# Autodesk Inventor assembly: EnglishAssembly
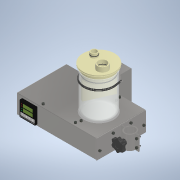
[picture p0: Inventor's stored thumbnail of the model, 180x180]
Saved by Autodesk Inventor 2020 (Build 240168000, 168)
## iProperties
Created: 2020-07-27
Part Number: EnglishAssembly
Document SubType Name: Assembly
Designer: Samuel
Author: Samuel
## Documents named in this file (31)
- C:\Users\Samuel\Desktop\EnglishAssembly.iam
- C:\Users\Samuel\Desktop\CNAF\CNAFgit\OpenHFNC\CAD\Prototype 3 (eng)\Box base_v7.ipt
- C:\Users\Samuel\Desktop\CNAF\CNAFgit\OpenHFNC\CAD\Prototype 3 (eng)\M4 Rivet nut.ipt
- C:\Users\Samuel\Desktop\CNAF\CNAFgit\OpenHFNC\CAD\Prototype 3 (eng)\RexC100 Temp control.ipt
- C:\Users\Samuel\Desktop\CNAF\CNAFgit\OpenHFNC\CAD\Prototype 3 (eng)\Switch OnOff 240V20A.ipt
- C:\Users\Samuel\Desktop\CNAF\CNAFgit\OpenHFNC\CAD\Prototype 3 (eng)\Solid State Rele SSR40DA.ipt
- C:\Users\Samuel\Desktop\CNAF\CNAFgit\OpenHFNC\CAD\Prototype 3 (eng)\Box top_v7.ipt
- C:\Users\Samuel\Desktop\CNAF\CNAFgit\OpenHFNC\CAD\Prototype 3 (eng)\Heater disk.ipt
- C:\Users\Samuel\Desktop\CNAF\CNAFgit\OpenHFNC\CAD\Prototype 3 (eng)\Oring 2-343.ipt
- C:\Users\Samuel\Desktop\CNAF\CNAFgit\OpenHFNC\CAD\Prototype 3 (eng)\Heater630W.ipt
- C:\Users\Samuel\Desktop\CNAF\CNAFgit\OpenHFNC\CAD\Prototype 3 (eng)\DIN912 M4x0.7x40-8.8 socket head screw.ipt
- C:\Users\Samuel\Desktop\CNAF\CNAFgit\OpenHFNC\CAD\Prototype 3 (eng)\DIN934-M4 nut.ipt
- C:\Users\Samuel\Desktop\CNAF\CNAFgit\OpenHFNC\CAD\Prototype 3 (eng)\DIN913-M5x5 socket screw flat end.ipt
- C:\Users\Samuel\Desktop\CNAF\CNAFgit\OpenHFNC\CAD\Prototype 3 (eng)\Thermocouple.ipt
- C:\Users\Samuel\Desktop\CNAF\CNAFgit\OpenHFNC\CAD\Prototype 3 (eng)\Heater Fixing Bar.ipt
- C:\Users\Samuel\Desktop\CNAF\CNAFgit\OpenHFNC\CAD\Prototype 3 (eng)\IEC C14 Male panel conector.ipt
- C:\Users\Samuel\Desktop\CNAF\CNAFgit\OpenHFNC\CAD\Prototype 3 (eng)\Precipitated Glass 600ml-De90-Di84-H120.ipt
- C:\Users\Samuel\Desktop\CNAF\CNAFgit\OpenHFNC\CAD\Prototype 3 (eng)\DIN912 M4x0.7x10-8.8 socket head screw.ipt
- C:\Users\Samuel\Desktop\CNAF\CNAFgit\OpenHFNC\CAD\Prototype 3 (eng)\DIN7991 M3x0.5x10-8.8 countersunk head cap screws.ipt
- C:\Users\Samuel\Desktop\CNAF\CNAFgit\OpenHFNC\CAD\Prototype 3 (eng)\Glass fixer plate.ipt
- C:\Users\Samuel\Desktop\CNAF\CNAFgit\OpenHFNC\CAD\Prototype 3 (eng)\Oring 2-159 Glass plate fixer.ipt
- C:\Users\Samuel\Desktop\CNAF\CNAFgit\OpenHFNC\CAD\Prototype 3 (eng)\Body glass top.ipt
- C:\Users\Samuel\Desktop\CNAF\CNAFgit\OpenHFNC\CAD\Prototype 3 (eng)\Oring 2-151 Deform.ipt
- C:\Users\Samuel\Desktop\CNAF\CNAFgit\OpenHFNC\CAD\Prototype 3 (eng)\DIN912 M4x0.7x16-8.8 socket head screw.ipt
- C:\Users\Samuel\Desktop\CNAF\CNAFgit\OpenHFNC\CAD\Prototype 3 (eng)\Corrugated-top connector.ipt
- C:\Users\Samuel\Desktop\CNAF\CNAFgit\OpenHFNC\CAD\Prototype 3 (eng)\Heated tube-top connector.ipt
- C:\Users\Samuel\Desktop\CNAF\CNAFgit\OpenHFNC\CAD\Prototype 3 (eng)\Oring 2-018 Deform.ipt
- C:\Users\Samuel\Desktop\CNAF\CNAFgit\OpenHFNC\CAD\Prototype 3 (eng)\Oring 2-022.ipt
- C:\Users\Samuel\Desktop\CNAF\CNAFgit\OpenHFNC\CAD\Prototype 3 (eng)\Paddle.ipt
- C:\Users\Samuel\Desktop\box-iv stand connector.iam
- C:\Users\Samuel\Desktop\CNAF\CNAFgit\OpenHFNC\CAD\Prototype 3 (eng)\Star Knob 1-4UNC.ipt
## Components (67 placed, 30 different names)
1. Box base_v7:1 — Cylindrical:1, Cylindrical:2, Cylindrical:3, Cylindrical:4, Cylindrical:5, Cylindrical:6, Cylindrical:7, Cylindrical:8, Rotational:1, Cylindrical:9, Rotational:2, Cylindrical:10, Cylindrical:11, Cylindrical:12, Rigid:1, Rigid:2, Rigid:3, Cylindrical:13, Rotational:7, Rotational:14
2. M4 Rivet nut:1 — Cylindrical:3
3. M4 Rivet nut:2 — Cylindrical:1
4. M4 Rivet nut:3 — Cylindrical:4
5. M4 Rivet nut:4 — Cylindrical:5
6. M4 Rivet nut:5 — Rotational:1
7. M4 Rivet nut:6 — Cylindrical:2
8. M4 Rivet nut:7 — Cylindrical:6
9. M4 Rivet nut:8 — Cylindrical:9
10. M4 Rivet nut:9 — Cylindrical:8
11. M4 Rivet nut:10 — Rotational:2
12. M4 Rivet nut:11 — Cylindrical:7
13. M4 Rivet nut:12 — Cylindrical:11
14. M4 Rivet nut:13 — Cylindrical:10
15. M4 Rivet nut:14 — Cylindrical:12
16. RexC100 Temp control:1 — Rigid:1
17. Switch OnOff 240V20A:1 — Rigid:2
18. SSR-XXDA:1 — Rigid:3
19. Box top_v7:1 — Cylindrical:13, Rotational:3, Cylindrical:15, Cylindrical:16, Cylindrical:20, Cylindrical:21, Rotational:9, Cylindrical:22, Cylindrical:23, Rotational:10, Rotational:11, Cylindrical:24, Rotational:17, Rotational:18, Cylindrical:30, Cylindrical:31
20. Heater disk:1 — Rotational:3, Rigid:4, Cylindrical:14, Rotational:4, Rotational:5, Cylindrical:17, Cylindrical:19, Rotational:8
21. Oring 2-343:1 — Rigid:4
22. Heater630W:1 — Cylindrical:14
23. DIN912 M4x0.7x40-8.8 socket head screw:1 — Cylindrical:15
24. DIN912 M4x0.7x40-8.8 socket head screw:2 — Cylindrical:16
25. DIN934-M4 nut:1 — Cylindrical:18
26. DIN934-M4 nut:2 — Rotational:6
27. DIN913-M5x5 socket screw flat end:1 — Rotational:4
28. DIN913-M5x5 socket screw flat end:2 — Rotational:5
29. Thermocouple:1 — Cylindrical:19
30. Heater Fixing Bar:1 — Cylindrical:17, Cylindrical:18, Rotational:6
31. IEC C14 Male panel conector:1 — Rotational:7, Rotational:12, Rotational:13
32. Precipitated Glass 600ml-De90-Di84-H120:1 — Rotational:8, Cylindrical:25, Cylindrical:26
33. DIN912 M4x0.7x10-8.8 socket head screw:1 — Cylindrical:21
34. DIN912 M4x0.7x10-8.8 socket head screw:2 — Cylindrical:20
35. DIN912 M4x0.7x10-8.8 socket head screw:3 — Cylindrical:22
36. DIN912 M4x0.7x10-8.8 socket head screw:4 — Rotational:16
37. DIN912 M4x0.7x10-8.8 socket head screw:5 — Rotational:18
38. DIN912 M4x0.7x10-8.8 socket head screw:6 — Rotational:15
39. DIN912 M4x0.7x10-8.8 socket head screw:7 — Rotational:11
40. DIN912 M4x0.7x10-8.8 socket head screw:9 — Cylindrical:23
41. DIN912 M4x0.7x10-8.8 socket head screw:10 — Rotational:9
42. DIN912 M4x0.7x10-8.8 socket head screw:11 — Cylindrical:24
43. DIN912 M4x0.7x10-8.8 socket head screw:12 — Rotational:17
44. DIN912 M4x0.7x10-8.8 socket head screw:14 — Rotational:10
45. DIN7991 M3x0.5x10-8.8 countersunk head cap screws:1 — Rotational:12
46. DIN7991 M3x0.5x10-8.8 countersunk head cap screws:2 — Rotational:13
47. Glass fixer plate:1 — Rotational:14, Rotational:15, Rotational:16
48. Oring 2-159 Glass plate fixer:1
49. Body glass top:1 — Cylindrical:25, Cylindrical:27, Cylindrical:28, Cylindrical:29, Rotational:19
50. Oring 2-151 Deform:1 — Cylindrical:26
51. DIN912 M4x0.7x16-8.8 socket head screw:1 — Cylindrical:27
52. Corrugated-top connector:1 — Cylindrical:29, Rigid:5
53. Heated tube-top connector:1 — Cylindrical:28, Rigid:6
54. Oring 2-018 Deform:1 — Rigid:5
55. Oring 2-022:1 — Rigid:6
56. Paddle:1 — Rotational:19
57. box-iv stand connector:1 [sub-assembly] — Cylindrical:30, Cylindrical:32, Cylindrical:33, Cylindrical:36, Cylindrical:37, Cylindrical:38
58. box-iv stand connector:2 [sub-assembly] — Cylindrical:31, Cylindrical:34, Cylindrical:35, Cylindrical:40, Cylindrical:41
59. Star Knob 1-4UNC:1 — Cylindrical:36
60. DIN912 M4x0.7x10-8.8 socket head screw:15 — Cylindrical:32
61. DIN912 M4x0.7x10-8.8 socket head screw:16 — Cylindrical:35
62. DIN912 M4x0.7x10-8.8 socket head screw:17 — Cylindrical:33
63. DIN912 M4x0.7x10-8.8 socket head screw:18 — Cylindrical:34
64. DIN912 M4x0.7x10-8.8 socket head screw:19 — Cylindrical:37
65. DIN912 M4x0.7x10-8.8 socket head screw:20 — Cylindrical:38
66. DIN934-M4 nut:4 — Cylindrical:40
67. DIN934-M4 nut:5 — Cylindrical:41
## Relationships (65: CylindricalJoint 40, RevoluteJoint 19, WeldJoint 6)
- Cylindrical:1: Box base_v7:1 ↔ M4 Rivet nut:2
- Cylindrical:2: Box base_v7:1 ↔ M4 Rivet nut:6
- Cylindrical:3: Box base_v7:1 ↔ M4 Rivet nut:1
- Cylindrical:4: Box base_v7:1 ↔ M4 Rivet nut:3
- Cylindrical:5: Box base_v7:1 ↔ M4 Rivet nut:4
- Cylindrical:6: Box base_v7:1 ↔ M4 Rivet nut:7
- Cylindrical:7: Box base_v7:1 ↔ M4 Rivet nut:11
- Cylindrical:8: Box base_v7:1 ↔ M4 Rivet nut:9
- Rotational:1 [RevoluteJoint]: Box base_v7:1 ↔ M4 Rivet nut:5
- Cylindrical:9: Box base_v7:1 ↔ M4 Rivet nut:8
- Rotational:2 [RevoluteJoint]: Box base_v7:1 ↔ M4 Rivet nut:10
- Cylindrical:10: Box base_v7:1 ↔ M4 Rivet nut:13
- Cylindrical:11: Box base_v7:1 ↔ M4 Rivet nut:12
- Cylindrical:12: Box base_v7:1 ↔ M4 Rivet nut:14
- Rigid:1 [WeldJoint]: Box base_v7:1 ↔ RexC100 Temp control:1
- Rigid:2 [WeldJoint]: Box base_v7:1 ↔ Switch OnOff 240V20A:1
- Rigid:3 [WeldJoint]: Box base_v7:1 ↔ SSR-XXDA:1
- Cylindrical:13: Box base_v7:1 ↔ Box top_v7:1
- Rotational:3 [RevoluteJoint]: Box top_v7:1 ↔ Heater disk:1
- Rigid:4 [WeldJoint]: Heater disk:1 ↔ Oring 2-343:1
- Cylindrical:14: Heater disk:1 ↔ Heater630W:1
- Cylindrical:15: Box top_v7:1 ↔ DIN912 M4x0.7x40-8.8 socket head screw:1
- Cylindrical:16: Box top_v7:1 ↔ DIN912 M4x0.7x40-8.8 socket head screw:2
- Rotational:4 [RevoluteJoint]: Heater disk:1 ↔ DIN913-M5x5 socket screw flat end:1
- Rotational:5 [RevoluteJoint]: Heater disk:1 ↔ DIN913-M5x5 socket screw flat end:2
- Cylindrical:17: Heater disk:1 ↔ Heater Fixing Bar:1
- Cylindrical:18: DIN934-M4 nut:1 ↔ Heater Fixing Bar:1
- Rotational:6 [RevoluteJoint]: DIN934-M4 nut:2 ↔ Heater Fixing Bar:1
- Cylindrical:19: Heater disk:1 ↔ Thermocouple:1
- Rotational:7 [RevoluteJoint]: Box base_v7:1 ↔ IEC C14 Male panel conector:1
- Rotational:8 [RevoluteJoint]: Heater disk:1 ↔ Precipitated Glass 600ml-De90-Di84-H120:1
- Cylindrical:20: Box top_v7:1 ↔ DIN912 M4x0.7x10-8.8 socket head screw:2
- Cylindrical:21: Box top_v7:1 ↔ DIN912 M4x0.7x10-8.8 socket head screw:1
- Rotational:9 [RevoluteJoint]: Box top_v7:1 ↔ DIN912 M4x0.7x10-8.8 socket head screw:10
- Cylindrical:22: Box top_v7:1 ↔ DIN912 M4x0.7x10-8.8 socket head screw:3
- Cylindrical:23: Box top_v7:1 ↔ DIN912 M4x0.7x10-8.8 socket head screw:9
- Rotational:10 [RevoluteJoint]: Box top_v7:1 ↔ DIN912 M4x0.7x10-8.8 socket head screw:14
- Rotational:11 [RevoluteJoint]: Box top_v7:1 ↔ DIN912 M4x0.7x10-8.8 socket head screw:7
- Rotational:12 [RevoluteJoint]: IEC C14 Male panel conector:1 ↔ DIN7991 M3x0.5x10-8.8 countersunk head cap screws:1
- Rotational:13 [RevoluteJoint]: IEC C14 Male panel conector:1 ↔ DIN7991 M3x0.5x10-8.8 countersunk head cap screws:2
- Rotational:14 [RevoluteJoint]: Box base_v7:1 ↔ Glass fixer plate:1
- Rotational:15 [RevoluteJoint]: DIN912 M4x0.7x10-8.8 socket head screw:6 ↔ Glass fixer plate:1
- Rotational:16 [RevoluteJoint]: DIN912 M4x0.7x10-8.8 socket head screw:4 ↔ Glass fixer plate:1
- Cylindrical:24: Box top_v7:1 ↔ DIN912 M4x0.7x10-8.8 socket head screw:11
- Rotational:17 [RevoluteJoint]: Box top_v7:1 ↔ DIN912 M4x0.7x10-8.8 socket head screw:12
- Rotational:18 [RevoluteJoint]: Box top_v7:1 ↔ DIN912 M4x0.7x10-8.8 socket head screw:5
- Cylindrical:25: Precipitated Glass 600ml-De90-Di84-H120:1 ↔ Body glass top:1
- Cylindrical:26: Precipitated Glass 600ml-De90-Di84-H120:1 ↔ Oring 2-151 Deform:1
- Cylindrical:27: Body glass top:1 ↔ DIN912 M4x0.7x16-8.8 socket head screw:1
- Cylindrical:28: Body glass top:1 ↔ Heated tube-top connector:1
- Cylindrical:29: Body glass top:1 ↔ Corrugated-top connector:1
- Rigid:5 [WeldJoint]: Corrugated-top connector:1 ↔ Oring 2-018 Deform:1
- Rigid:6 [WeldJoint]: Heated tube-top connector:1 ↔ Oring 2-022:1
- Rotational:19 [RevoluteJoint]: Body glass top:1 ↔ Paddle:1
- Cylindrical:30: Box top_v7:1 ↔ box-iv stand connector:1
- Cylindrical:31: Box top_v7:1 ↔ box-iv stand connector:2
- Cylindrical:32: box-iv stand connector:1 ↔ DIN912 M4x0.7x10-8.8 socket head screw:15
- Cylindrical:33: box-iv stand connector:1 ↔ DIN912 M4x0.7x10-8.8 socket head screw:17
- Cylindrical:34: box-iv stand connector:2 ↔ DIN912 M4x0.7x10-8.8 socket head screw:18
- Cylindrical:35: box-iv stand connector:2 ↔ DIN912 M4x0.7x10-8.8 socket head screw:16
- Cylindrical:36: box-iv stand connector:1 ↔ Star Knob 1-4UNC:1
- Cylindrical:37: box-iv stand connector:1 ↔ DIN912 M4x0.7x10-8.8 socket head screw:19
- Cylindrical:38: box-iv stand connector:1 ↔ DIN912 M4x0.7x10-8.8 socket head screw:20
- Cylindrical:40: box-iv stand connector:2 ↔ DIN934-M4 nut:4
- Cylindrical:41: box-iv stand connector:2 ↔ DIN934-M4 nut:5
